# Autodesk Inventor assembly: J005108
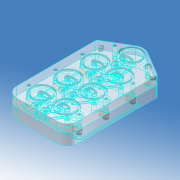
[picture p0: Inventor's stored thumbnail of the model, 180x180]
Saved by Autodesk Inventor 2015 SP1 (Build 190203100, 203)
## iProperties
RuleStatus: InUse
AfterDocSave0: file://Part Number Cleaner
Created: 2015-03-14
Vendor: HHMI: JRC - ID&F
Document SubType Name: Assembly
Designer: JORDANJ
Project: P-171601
Part Number: J005108
Description: COMPONENT OF AN AUTOMATED LIQUID HANDLING MACHINE SPECIFICALLY DESIGNED FOR THE IN SITU RNA HYBRIDIZATION OF DROSOPHILA EMBRYOS
DESIGN DEPARTMENT: HHMI: JRC - ID&F
LAB/DEPT: STERN (LAB)
REQUESTING SCIENTIST: STERN, DAVID
SPECIAL FINISH: POLISH CLEAR
SURFACE ROUGHNESS: 32 Ra
ALTERED ITEM PART NUMBER: N/A
ALTERED ITEM VENDOR: N/A
ALTERED ITEM DESCRIPTION: N/A
Revision Number: A
## Documents named in this file (5)
- C:\_WORKSPACE\DATA\PROJECTS\HYBRIDIZER\MCAD\MICROPLATE\24W DISPENSE MANIFOLD ASSY.iam
- C:\_WORKSPACE\DATA\PROJECTS\HYBRIDIZER\MCAD\MICROPLATE\24W DISPENSE MANIFOLD.ipt
- C:\_WORKSPACE\DATA\Imported Components\20150305-185214-24176534\PEM ISC-440.ipt
- C:\_WORKSPACE\DATA\PROJECTS\HYBRIDIZER\MCAD\MICROPLATE\_24W.ipt
- C:\_WORKSPACE\DATA\Imported Components\20150327-142204-70136782\PEM ISC-832.ipt
## Components (19 placed, 3 different names)
1. 24W DISPENSE MANIFOLD:1 — Insert:13, Insert:14, Insert:15, Insert:16
2. PEM ISC-440:7
3. PEM ISC-440:8
4. PEM ISC-440:9
5. PEM ISC-440:10
6. PEM ISC-832:1 — Insert:13
7. PEM ISC-832:2 — Insert:14
8. PEM ISC-832:4 — Insert:16
9. PEM ISC-440:2
10. PEM ISC-440:1
11. PEM ISC-832:3 — Insert:15
12. PEM ISC-832:5
13. PEM ISC-440:11
14. PEM ISC-440:12
15. PEM ISC-832:6
16. PEM ISC-832:7
17. PEM ISC-440:13
18. PEM ISC-440:14
19. PEM ISC-832:8
## Component patterns: (3 elements, first: PEM ISC-832:4 + PEM ISC-440:2 + PEM ISC-440:1 + PEM ISC-832:3)
## Relationships (10: Insert 10)
- [Insert]: 24W DISPENSE MANIFOLD:1 ↔ PEM ISC-440:1
- [Insert]: 24W DISPENSE MANIFOLD:1 ↔ PEM ISC-440:2
- [Insert]: 24W DISPENSE MANIFOLD:1 ↔ PEM ISC-440:7
- [Insert]: 24W DISPENSE MANIFOLD:1 ↔ PEM ISC-440:8
- [Insert]: 24W DISPENSE MANIFOLD:1 ↔ PEM ISC-440:9
- [Insert]: 24W DISPENSE MANIFOLD:1 ↔ PEM ISC-440:10
- Insert:13: 24W DISPENSE MANIFOLD:1 ↔ PEM ISC-832:1
- Insert:14: 24W DISPENSE MANIFOLD:1 ↔ PEM ISC-832:2
- Insert:15: 24W DISPENSE MANIFOLD:1 ↔ PEM ISC-832:3
- Insert:16: 24W DISPENSE MANIFOLD:1 ↔ PEM ISC-832:4
## Named parameters: microplate_well_no_x = 4, microplate_well_spacing = 18.78071 mm, microplate_well_no_z = 6
